# Autodesk Inventor assembly: robot_frame_layer1-evan
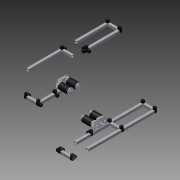
[picture p0: Inventor's stored thumbnail of the model, 180x180]
Saved by Autodesk Inventor 2011 SP1 (Build 150282100, 282)
## iProperties
Created: 2013-01-17
Part Number: robot_frame_layer1-evan
Document SubType Name: Assembly
Designer: Christopher
Author: Christopher
## Documents named in this file (12)
- \\WW427-DATA1\StuHome\971065\Documents\GitHub\Robotics 2112 Yes 2112\2013CAD\2013 robot\Spiderbot\robot_frame_layer1-evan.iam
- \\WW427-DATA1\StuHome\971065\Documents\GitHub\Robotics 2112 Yes 2112\2013CAD\2013 robot\forklift\robot parts\1tube_4_layer1_outside.ipt
- \\WW427-DATA1\StuHome\971065\Documents\GitHub\Robotics 2112 Yes 2112\2013CAD\2013 robot\forklift\robot parts\1tube_6_layer1_boardsupportsupport.ipt
- \\WW427-DATA1\StuHome\971065\Documents\GitHub\Robotics 2112 Yes 2112\2013CAD\2013 robot\forklift\robot parts\1tube_6_layer1_motorsupport.ipt
- \\WW427-DATA1\StuHome\971065\Documents\GitHub\Robotics 2112 Yes 2112\2013CAD\2013 robot\forklift\robot parts\1tube_14_layer1_inside.ipt
- \\WW427-DATA1\StuHome\971065\Documents\GitHub\Robotics 2112 Yes 2112\2013CAD\2013 robot\forklift\Misc parts\3-way corner.ipt
- \\WW427-DATA1\StuHome\971065\Documents\GitHub\Robotics 2112 Yes 2112\2013CAD\2013 robot\forklift\Misc parts\4-way corner.ipt
- \\WW427-DATA1\StuHome\971065\Documents\GitHub\Robotics 2112 Yes 2112\2013CAD\2013 robot\forklift\Misc parts\5-way corner.ipt
- \\WW427-DATA1\StuHome\971065\Documents\GitHub\Robotics 2112 Yes 2112\2013CAD\2013 robot\forklift\robot parts\1tube_13_layer1_side.ipt
- \\WW427-DATA1\StuHome\971065\Documents\GitHub\Robotics 2112 Yes 2112\2013CAD\2013 robot\forklift\Chassis\Chassis_CIMGearbox_AndyMark_am-0734.ipt
- \\WW427-DATA1\StuHome\971065\Documents\GitHub\Robotics 2112 Yes 2112\2013CAD\2013 robot\forklift\Misc parts\nut_.25_20.ipt
- \\WW427-DATA1\StuHome\971065\Documents\GitHub\Robotics 2112 Yes 2112\2013CAD\2013 robot\forklift\frame parts\corner_prop.ipt
## Components (41 placed, 11 different names)
1. 1tube_4_layer1_outside:1 — Mate:7, Mate:8, Mate:9, Mate:10, Mate:11, Mate:12
2. 1tube_6_layer1_boardsupportsupport:1 — Mate:22, Mate:23, Mate:24, Mate:25, Mate:26, Mate:27
3. 1tube_6_layer1_motorsupport:1 — Mate:28, Mate:29, Mate:30, Mate:110, Flush:1, Mate:120, Flush:2
4. 3-way corner:1 — Mate:13, Mate:14, Mate:15, Mate:150, Mate:151
5. 3-way corner:2 — Mate:7, Mate:8, Mate:9, Mate:148
6. 3-way corner:4 — Mate:70, Mate:71, Mate:72, Mate:121, Mate:122, Mate:131
7. 3-way corner:5 — Mate:73, Mate:74, Mate:75, Mate:152, Flush:12, Flush:13, Mate:153
8. 3-way corner:6 — Mate:67, Mate:68, Mate:69, Flush:8, Flush:9
9. 3-way corner:7 — Mate:16, Mate:17, Mate:18, Mate:142, Mate:143, Mate:144
10. 4-way corner:2 — Mate:10, Mate:11, Mate:12, Mate:22, Mate:23, Mate:24
11. 1tube_4_layer1_outside:2 — Mate:13, Mate:14, Mate:15, Mate:16, Mate:17, Mate:18
12. 4-way corner:3 — Mate:25, Mate:26, Mate:27, Mate:28, Mate:29, Mate:30
13. 4-way corner:5 — Mate:53, Mate:54, Mate:128, Mate:129, Mate:130
14. 4-way corner:6 — Mate:52, Mate:64, Mate:65, Mate:66
15. 1tube_6_layer1_motorsupport:2 — Mate:127, Flush:4, Flush:5, Mate:128, Mate:129, Mate:130, Mate:135, Mate:136, Mate:137
16. 1tube_6_layer1_boardsupportsupport:2 — Mate:52, Mate:53, Mate:54
17. 1tube_4_layer1_outside:3 — Mate:64, Mate:65, Mate:66, Mate:67, Mate:68, Mate:69
18. 1tube_4_layer1_outside:4 — Mate:70, Mate:71, Mate:72, Mate:73, Mate:74, Mate:75
19. 5-way corner:1 — Mate:85, Mate:86, Mate:87, Mate:123, Mate:124, Mate:125, Mate:126, Mate:135, Mate:136, Mate:137
20. 5-way corner:2 — Mate:110, Mate:116, Mate:139, Mate:140, Mate:141, Mate:147
21. 1tube_4_layer1_outside:5 — Mate:85, Mate:86, Mate:87, Mate:88, Mate:89, Mate:90
22. 4-way corner:7 — Mate:88, Mate:89, Mate:90, Mate:138, Flush:6, Flush:7
23. 4-way corner:8 — Mate:114, Mate:115, Mate:145, Flush:10, Flush:11, Mate:146, Mate:149
24. 1tube_4_layer1_outside:6 — Mate:114, Mate:115, Mate:116, Mate:146, Mate:147
25. Chassis_CIMGearbox_AndyMark_am-0734:1 — Flush:1, Mate:120, Flush:2
26. Chassis_CIMGearbox_AndyMark_am-0734:2 — Mate:127, Flush:4, Flush:5
27. 1tube_13_layer1_side:3 — Mate:121, Mate:122, Mate:123, Mate:124, Mate:125, Mate:126, Mate:131, Insert:11, Insert:12
28. 1tube_13_layer1_side:4 — Mate:152, Flush:12, Flush:13, Mate:153, Insert:31, Insert:32
29. 1tube_14_layer1_inside:2 — Mate:138, Flush:6, Flush:7, Flush:8, Flush:9
30. 1tube_14_layer1_inside:3 — Mate:145, Flush:10, Flush:11, Mate:148
31. 1tube_13_layer1_side:5 — Mate:139, Mate:140, Mate:141, Mate:142, Mate:143, Mate:144, Insert:9, Insert:10
32. 1tube_13_layer1_side:6 — Mate:149, Mate:150, Mate:151, Insert:33, Insert:34
33. nut_.25_20:1 — Insert:9
34. nut_.25_20:2 — Insert:10
35. nut_.25_20:3 — Insert:12
36. nut_.25_20:4 — Insert:11
37. nut_.25_20:5 — Insert:32
38. nut_.25_20:6 — Insert:31
39. nut_.25_20:7 — Insert:34
40. nut_.25_20:8 — Insert:33
41. corner_prop:1
## Relationships (97: Mate 77, Flush 12, Insert 8)
- Mate:7: 1tube_4_layer1_outside:1 ↔ 3-way corner:2
- Mate:8: 1tube_4_layer1_outside:1 ↔ 3-way corner:2
- Mate:9: 1tube_4_layer1_outside:1 ↔ 3-way corner:2
- Mate:10: 1tube_4_layer1_outside:1 ↔ 4-way corner:2
- Mate:11: 1tube_4_layer1_outside:1 ↔ 4-way corner:2
- Mate:12: 1tube_4_layer1_outside:1 ↔ 4-way corner:2
- Mate:13: 3-way corner:1 ↔ 1tube_4_layer1_outside:2
- Mate:14: 3-way corner:1 ↔ 1tube_4_layer1_outside:2
- Mate:15: 3-way corner:1 ↔ 1tube_4_layer1_outside:2
- Mate:16: 3-way corner:7 ↔ 1tube_4_layer1_outside:2
- Mate:17: 3-way corner:7 ↔ 1tube_4_layer1_outside:2
- Mate:18: 3-way corner:7 ↔ 1tube_4_layer1_outside:2
- Mate:22: 1tube_6_layer1_boardsupportsupport:1 ↔ 4-way corner:2
- Mate:23: 1tube_6_layer1_boardsupportsupport:1 ↔ 4-way corner:2
- Mate:24: 1tube_6_layer1_boardsupportsupport:1 ↔ 4-way corner:2
- Mate:25: 1tube_6_layer1_boardsupportsupport:1 ↔ 4-way corner:3
- Mate:26: 1tube_6_layer1_boardsupportsupport:1 ↔ 4-way corner:3
- Mate:27: 1tube_6_layer1_boardsupportsupport:1 ↔ 4-way corner:3
- Mate:28: 1tube_6_layer1_motorsupport:1 ↔ 4-way corner:3
- Mate:29: 1tube_6_layer1_motorsupport:1 ↔ 4-way corner:3
- Mate:30: 1tube_6_layer1_motorsupport:1 ↔ 4-way corner:3
- Mate:52: 4-way corner:6 ↔ 1tube_6_layer1_boardsupportsupport:2
- Mate:53: 4-way corner:5 ↔ 1tube_6_layer1_boardsupportsupport:2
- Mate:54: 4-way corner:5 ↔ 1tube_6_layer1_boardsupportsupport:2
- Mate:64: 4-way corner:6 ↔ 1tube_4_layer1_outside:3
- Mate:65: 4-way corner:6 ↔ 1tube_4_layer1_outside:3
- Mate:66: 4-way corner:6 ↔ 1tube_4_layer1_outside:3
- Mate:67: 3-way corner:6 ↔ 1tube_4_layer1_outside:3
- Mate:68: 3-way corner:6 ↔ 1tube_4_layer1_outside:3
- Mate:69: 3-way corner:6 ↔ 1tube_4_layer1_outside:3
- Mate:70: 3-way corner:4 ↔ 1tube_4_layer1_outside:4
- Mate:71: 3-way corner:4 ↔ 1tube_4_layer1_outside:4
- Mate:72: 3-way corner:4 ↔ 1tube_4_layer1_outside:4
- Mate:73: 3-way corner:5 ↔ 1tube_4_layer1_outside:4
- Mate:74: 3-way corner:5 ↔ 1tube_4_layer1_outside:4
- Mate:75: 3-way corner:5 ↔ 1tube_4_layer1_outside:4
- Mate:85: 5-way corner:1 ↔ 1tube_4_layer1_outside:5
- Mate:86: 5-way corner:1 ↔ 1tube_4_layer1_outside:5
- Mate:87: 5-way corner:1 ↔ 1tube_4_layer1_outside:5
- Mate:88: 1tube_4_layer1_outside:5 ↔ 4-way corner:7
- Mate:89: 1tube_4_layer1_outside:5 ↔ 4-way corner:7
- Mate:90: 1tube_4_layer1_outside:5 ↔ 4-way corner:7
- Mate:110: 1tube_6_layer1_motorsupport:1 ↔ 5-way corner:2
- Mate:114: 4-way corner:8 ↔ 1tube_4_layer1_outside:6
- Mate:115: 4-way corner:8 ↔ 1tube_4_layer1_outside:6
- Mate:116: 5-way corner:2 ↔ 1tube_4_layer1_outside:6
- Flush:1: 1tube_6_layer1_motorsupport:1 ↔ Chassis_CIMGearbox_AndyMark_am-0734:1
- Mate:120: 1tube_6_layer1_motorsupport:1 ↔ Chassis_CIMGearbox_AndyMark_am-0734:1
- Mate:121: 3-way corner:4 ↔ 1tube_13_layer1_side:3
- Mate:122: 3-way corner:4 ↔ 1tube_13_layer1_side:3
- Mate:123: 5-way corner:1 ↔ 1tube_13_layer1_side:3
- Mate:124: 5-way corner:1 ↔ 1tube_13_layer1_side:3
- Mate:125: 5-way corner:1 ↔ 1tube_13_layer1_side:3
- Mate:126: 5-way corner:1 ↔ 1tube_13_layer1_side:3
- Flush:2: 1tube_6_layer1_motorsupport:1 ↔ Chassis_CIMGearbox_AndyMark_am-0734:1
- Mate:127: 1tube_6_layer1_motorsupport:2 ↔ Chassis_CIMGearbox_AndyMark_am-0734:2
- Flush:4: 1tube_6_layer1_motorsupport:2 ↔ Chassis_CIMGearbox_AndyMark_am-0734:2
- Flush:5: 1tube_6_layer1_motorsupport:2 ↔ Chassis_CIMGearbox_AndyMark_am-0734:2
- Mate:128: 4-way corner:5 ↔ 1tube_6_layer1_motorsupport:2
- Mate:129: 4-way corner:5 ↔ 1tube_6_layer1_motorsupport:2
- Mate:130: 4-way corner:5 ↔ 1tube_6_layer1_motorsupport:2
- Mate:131: 3-way corner:4 ↔ 1tube_13_layer1_side:3
- Mate:135: 1tube_6_layer1_motorsupport:2 ↔ 5-way corner:1
- Mate:136: 1tube_6_layer1_motorsupport:2 ↔ 5-way corner:1
- Mate:137: 1tube_6_layer1_motorsupport:2 ↔ 5-way corner:1
- Mate:138: 4-way corner:7 ↔ 1tube_14_layer1_inside:2
- Flush:6: 4-way corner:7 ↔ 1tube_14_layer1_inside:2
- Flush:7: 4-way corner:7 ↔ 1tube_14_layer1_inside:2
- Flush:8: 3-way corner:6 ↔ 1tube_14_layer1_inside:2
- Flush:9: 3-way corner:6 ↔ 1tube_14_layer1_inside:2
- Mate:139: 5-way corner:2 ↔ 1tube_13_layer1_side:5
- Mate:140: 5-way corner:2 ↔ 1tube_13_layer1_side:5
- Mate:141: 5-way corner:2 ↔ 1tube_13_layer1_side:5
- Mate:142: 3-way corner:7 ↔ 1tube_13_layer1_side:5
- Mate:143: 3-way corner:7 ↔ 1tube_13_layer1_side:5
- Mate:144: 3-way corner:7 ↔ 1tube_13_layer1_side:5
- Mate:145: 4-way corner:8 ↔ 1tube_14_layer1_inside:3
- Flush:10: 4-way corner:8 ↔ 1tube_14_layer1_inside:3
- Flush:11: 4-way corner:8 ↔ 1tube_14_layer1_inside:3
- Mate:146: 4-way corner:8 ↔ 1tube_4_layer1_outside:6
- Mate:147: 5-way corner:2 ↔ 1tube_4_layer1_outside:6
- Mate:148: 3-way corner:2 ↔ 1tube_14_layer1_inside:3
- Mate:149: 4-way corner:8 ↔ 1tube_13_layer1_side:6
- Mate:150: 3-way corner:1 ↔ 1tube_13_layer1_side:6
- Mate:151: 3-way corner:1 ↔ 1tube_13_layer1_side:6
- Mate:152: 3-way corner:5 ↔ 1tube_13_layer1_side:4
- Flush:12: 3-way corner:5 ↔ 1tube_13_layer1_side:4
- Flush:13: 3-way corner:5 ↔ 1tube_13_layer1_side:4
- Mate:153: 3-way corner:5 ↔ 1tube_13_layer1_side:4
- Insert:9: 1tube_13_layer1_side:5 ↔ nut_.25_20:1
- Insert:10: 1tube_13_layer1_side:5 ↔ nut_.25_20:2
- Insert:11: 1tube_13_layer1_side:3 ↔ nut_.25_20:4
- Insert:12: 1tube_13_layer1_side:3 ↔ nut_.25_20:3
- Insert:31: 1tube_13_layer1_side:4 ↔ nut_.25_20:6
- Insert:32: 1tube_13_layer1_side:4 ↔ nut_.25_20:5
- Insert:33: 1tube_13_layer1_side:6 ↔ nut_.25_20:8
- Insert:34: 1tube_13_layer1_side:6 ↔ nut_.25_20:7
